# Autodesk Inventor assembly: hipjoint_toleg_right
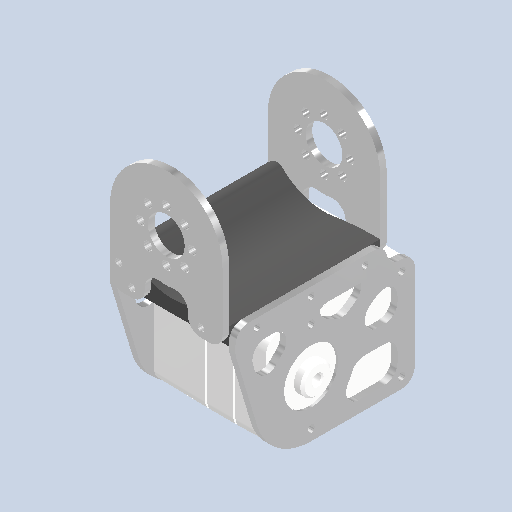
[picture p0: Inventor's stored thumbnail of the model, 512x512]
Saved by Autodesk Inventor 2024.1 (Build 281209000, 209)
## iProperties
Created: 2024-02-12
Part Number: hipjoint_toleg_right
Document SubType Name: Assembly
Designer: hibik
Author: hibik
## Documents named in this file (5)
- C:\Users\hibik\Desktop\ロボメカ\HR\2024.02.11 Rl\02.11 ProtType\hipjoint_toleg_right.iam
- C:\Users\hibik\Desktop\ロボメカ\HR\2024.02.11 Rl\02.11 ProtType\hipjoint_toleg_middle.ipt
- C:\Users\hibik\Desktop\ロボメカ\HR\2024.02.11 Rl\02.11 ProtType\hipjoint_toleg_upper.ipt
- C:\Users\hibik\Desktop\ロボメカ\HR\2024.02.11 Rl\02.11 ProtType\hipjoint_toleg_under.ipt
- C:\Users\hibik\Desktop\ロボメカ\HR\2024.02.11 Rl\KRS3300モータ.ipt
## Components (6 placed, 4 different names)
1. hipjoint_toleg_middle:1 — メイト:1, メイト:2, フラッシュ:1, フラッシュ:2, フラッシュ:3, フラッシュ:4, フラッシュ:5, フラッシュ:6, メイト:3, メイト:4, 挿入:1, 挿入:2
2. hipjoint_toleg_upper:1 — メイト:2, フラッシュ:1, フラッシュ:4
3. hipjoint_toleg_upper:2 — メイト:1, フラッシュ:2, フラッシュ:3
4. hipjoint_toleg_under:1 — フラッシュ:6, メイト:3, 挿入:1, 挿入:3, 角度:1
5. hipjoint_toleg_under:2 — フラッシュ:5, メイト:4, 挿入:2
6. KRS3300モータ:1 — 挿入:3, 角度:1
## Relationships (14: Flush 6, Mate 4, Insert 3, Angle 1)
- メイト:1 [Mate]: hipjoint_toleg_middle:1 ↔ hipjoint_toleg_upper:2
- メイト:2 [Mate]: hipjoint_toleg_middle:1 ↔ hipjoint_toleg_upper:1
- フラッシュ:1 [Flush]: hipjoint_toleg_middle:1 ↔ hipjoint_toleg_upper:1
- フラッシュ:2 [Flush]: hipjoint_toleg_middle:1 ↔ hipjoint_toleg_upper:2
- フラッシュ:3 [Flush]: hipjoint_toleg_middle:1 ↔ hipjoint_toleg_upper:2
- フラッシュ:4 [Flush]: hipjoint_toleg_middle:1 ↔ hipjoint_toleg_upper:1
- フラッシュ:5 [Flush]: hipjoint_toleg_middle:1 ↔ hipjoint_toleg_under:2
- フラッシュ:6 [Flush]: hipjoint_toleg_middle:1 ↔ hipjoint_toleg_under:1
- メイト:3 [Mate]: hipjoint_toleg_middle:1 ↔ hipjoint_toleg_under:1
- メイト:4 [Mate]: hipjoint_toleg_middle:1 ↔ hipjoint_toleg_under:2
- 挿入:1 [Insert]: hipjoint_toleg_middle:1 ↔ hipjoint_toleg_under:1
- 挿入:2 [Insert]: hipjoint_toleg_middle:1 ↔ hipjoint_toleg_under:2
- 挿入:3 [Insert]: hipjoint_toleg_under:1 ↔ KRS3300モータ:1
- 角度:1 [Angle] (0 deg): hipjoint_toleg_under:1 ↔ KRS3300モータ:1
